# Autodesk Inventor assembly: Assemlby_lightsheet_generator_passive_v2
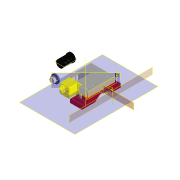
[picture p0: Inventor's stored thumbnail of the model, 180x180]
Saved by Autodesk Inventor 2022 (Build 260153000, 153)
## iProperties
Created: 2022-12-16
Part Number: Assemlby_lightsheet_generator_passive_v2
Document SubType Name: Assembly
Designer: UC2
Author: UC2
## Documents named in this file (7)
- C:\Users\diederichbenedict\Dropbox\Dokumente\Promotion\PROJECTS\HoLiSheet\INVENTOR\Assemlby_lightsheet_generator_passive_v2.iam
- C:\Users\diederichbenedict\Dropbox\Dokumente\Promotion\PROJECTS\HoLiSheet\INVENTOR\00_CCTV_lens_M12_25mm_5mp.ipt
- C:\Users\diederichbenedict\Dropbox\Dokumente\Promotion\PROJECTS\HoLiSheet\INVENTOR\00_Thorlabs_LJ1878L1-A-Step.ipt
- C:\Users\diederichbenedict\Dropbox\Dokumente\Promotion\PROJECTS\HoLiSheet\INVENTOR\00_SMAConnector_fiber copy.ipt
- C:\Users\diederichbenedict\Dropbox\Dokumente\Promotion\PROJECTS\HoLiSheet\INVENTOR\30_Lightsheet_generator_passive_base_v1.ipt
- C:\Users\diederichbenedict\Dropbox\Dokumente\Promotion\PROJECTS\HoLiSheet\INVENTOR\30_Lightsheet_generator_passive_lid_v1.ipt
- C:\Users\diederichbenedict\Dropbox\Dokumente\Promotion\PROJECTS\HoLiSheet\INVENTOR\30_Laser_to_M12Adapter.ipt
## Components (6 placed, 6 different names)
1. 30_Lightsheet_generator_passive_lid_v1:1 — Fluchtend:7, Fluchtend:8, Passend:1, Fluchtend:9, Fluchtend:10, Passend:4, Einfügen:2, Einfügen:3, Fluchtend:12
2. 00_Thorlabs_LJ1878L1-A-Step:1 — Fluchtend:7, Fluchtend:8, Fluchtend:9, Fluchtend:10
3. 30_Lightsheet_generator_passive_base_v1:1 — Einfügen:2, Einfügen:3, Fluchtend:12, Winkel:2, Passend:7, Fluchtend:13
4. 30_Laser_to_M12Adapter:1 — Winkel:2, Passend:7, Fluchtend:13
5. 00_CCTV_lens_M12_25mm_5mp:1
6. 00_SMAConnector_fiber copy:1
## Relationships (15: Flush 6, Mate 5, Angle 2, Insert 2)
- Fluchtend:7 [Flush] (1 mm): 30_Lightsheet_generator_passive_lid_v1:1 ↔ 00_Thorlabs_LJ1878L1-A-Step:1
- Fluchtend:8 [Flush]: 30_Lightsheet_generator_passive_lid_v1:1 ↔ 00_Thorlabs_LJ1878L1-A-Step:1
- Passend:1 [Mate]: 30_Lightsheet_generator_passive_lid_v1:1
- Fluchtend:9 [Flush]: 30_Lightsheet_generator_passive_lid_v1:1 ↔ 00_Thorlabs_LJ1878L1-A-Step:1
- Fluchtend:10 [Flush]: 30_Lightsheet_generator_passive_lid_v1:1 ↔ 00_Thorlabs_LJ1878L1-A-Step:1
- Passend:4 [Mate]: 30_Lightsheet_generator_passive_lid_v1:1
- Passend:5 [Mate]
- Passend:6 [Mate]
- Winkel:1 [Angle] (90 deg)
- Einfügen:2 [Insert]: 30_Lightsheet_generator_passive_lid_v1:1 ↔ 30_Lightsheet_generator_passive_base_v1:1
- Einfügen:3 [Insert]: 30_Lightsheet_generator_passive_lid_v1:1 ↔ 30_Lightsheet_generator_passive_base_v1:1
- Fluchtend:12 [Flush]: 30_Lightsheet_generator_passive_lid_v1:1 ↔ 30_Lightsheet_generator_passive_base_v1:1
- Winkel:2 [Angle] (270 deg): 30_Lightsheet_generator_passive_base_v1:1 ↔ 30_Laser_to_M12Adapter:1
- Passend:7 [Mate]: 30_Lightsheet_generator_passive_base_v1:1 ↔ 30_Laser_to_M12Adapter:1
- Fluchtend:13 [Flush] (3.5 mm): 30_Lightsheet_generator_passive_base_v1:1 ↔ 30_Laser_to_M12Adapter:1
